(part 1 of 2)
# Autodesk Inventor assembly: DesignRootModel^PCB_ESP32-C3-MINI-1_V1(2)_PCB_ESP32-C3-MINI-1_V1
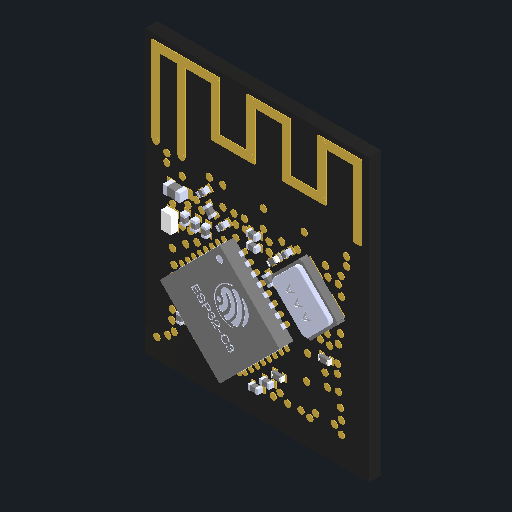
[picture p0: Inventor's stored thumbnail of the model, 512x512]
Saved by Autodesk Inventor 2026.2 (Build 302298000, 298)
## iProperties
Created: 2025-12-23
Part Number: DesignRootModel^PCB_ESP32-C3-MINI-1_V1(2)_PCB_ESP32-C3-MINI-1_V1
Document SubType Name: Assembly
Designer: test
Author: test
## Documents named in this file (333)
- D:\Projects\WearableWLED\WearableWLED_Mechanical\board\WearableWLED_Hardware\WearableWLED_Hardware\DesignRootModel^PCB_ESP32-C3-MINI-1_V1(2)_PCB_ESP32-C3-MINI-1_V1.iam
- D:\Projects\WearableWLED\WearableWLED_Mechanical\board\WearableWLED_Hardware\WearableWLED_Hardware\Submodel-SOD882_part^DesignRootModel_PCB_ESP32-C3-MINI-1_V1(2)_PCB_ESP32-C3-MINI-1_V1.iam
- D:\Projects\WearableWLED\WearableWLED_Mechanical\board\WearableWLED_Hardware\WearableWLED_Hardware\Submodel-R0201_part^DesignRootModel_PCB_ESP32-C3-MINI-1_V1(2)_PCB_ESP32-C3-MINI-1_V1.iam
- D:\Projects\WearableWLED\WearableWLED_Mechanical\board\WearableWLED_Hardware\WearableWLED_Hardware\Submodel-MINI-ANT-TYPED-H_1968823293_part^DesignRootModel_PCB_ESP32-C3-MINI-1_V1(2)_PCB_ESP32-C3-MIN.iam
- D:\Projects\WearableWLED\WearableWLED_Mechanical\board\WearableWLED_Hardware\WearableWLED_Hardware\Submodel-C0402_part^DesignRootModel_PCB_ESP32-C3-MINI-1_V1(2)_PCB_ESP32-C3-MINI-1_V1.iam
- D:\Projects\WearableWLED\WearableWLED_Mechanical\board\WearableWLED_Hardware\WearableWLED_Hardware\Submodel-R0201_part^DesignRootModel_PCB_ESP32-C3-MINI-1_V1(2)_PCB_ESP32-C3-MINI-1_V1_1.iam
- D:\Projects\WearableWLED\WearableWLED_Mechanical\board\WearableWLED_Hardware\WearableWLED_Hardware\Submodel-C0201_part^DesignRootModel_PCB_ESP32-C3-MINI-1_V1(2)_PCB_ESP32-C3-MINI-1_V1.iam
- D:\Projects\WearableWLED\WearableWLED_Mechanical\board\WearableWLED_Hardware\WearableWLED_Hardware\Submodel-R0201_part^DesignRootModel_PCB_ESP32-C3-MINI-1_V1(2)_PCB_ESP32-C3-MINI-1_V1_2.iam
- D:\Projects\WearableWLED\WearableWLED_Mechanical\board\WearableWLED_Hardware\WearableWLED_Hardware\Submodel-C0201_part^DesignRootModel_PCB_ESP32-C3-MINI-1_V1(2)_PCB_ESP32-C3-MINI-1_V1_1.iam
- D:\Projects\WearableWLED\WearableWLED_Mechanical\board\WearableWLED_Hardware\WearableWLED_Hardware\Submodel-C0201_part^DesignRootModel_PCB_ESP32-C3-MINI-1_V1(2)_PCB_ESP32-C3-MINI-1_V1_2.iam
- D:\Projects\WearableWLED\WearableWLED_Mechanical\board\WearableWLED_Hardware\WearableWLED_Hardware\Submodel-C0201_part^DesignRootModel_PCB_ESP32-C3-MINI-1_V1(2)_PCB_ESP32-C3-MINI-1_V1_3.iam
- D:\Projects\WearableWLED\WearableWLED_Mechanical\board\WearableWLED_Hardware\WearableWLED_Hardware\Submodel-C0201_part^DesignRootModel_PCB_ESP32-C3-MINI-1_V1(2)_PCB_ESP32-C3-MINI-1_V1_4.iam
- D:\Projects\WearableWLED\WearableWLED_Mechanical\board\WearableWLED_Hardware\WearableWLED_Hardware\Submodel-C0201_part^DesignRootModel_PCB_ESP32-C3-MINI-1_V1(2)_PCB_ESP32-C3-MINI-1_V1_5.iam
- D:\Projects\WearableWLED\WearableWLED_Mechanical\board\WearableWLED_Hardware\WearableWLED_Hardware\Submodel-C0201_part^DesignRootModel_PCB_ESP32-C3-MINI-1_V1(2)_PCB_ESP32-C3-MINI-1_V1_6.iam
- D:\Projects\WearableWLED\WearableWLED_Mechanical\board\WearableWLED_Hardware\WearableWLED_Hardware\Submodel-C0201_part^DesignRootModel_PCB_ESP32-C3-MINI-1_V1(2)_PCB_ESP32-C3-MINI-1_V1_7.iam
- D:\Projects\WearableWLED\WearableWLED_Mechanical\board\WearableWLED_Hardware\WearableWLED_Hardware\Submodel-C0201_part^DesignRootModel_PCB_ESP32-C3-MINI-1_V1(2)_PCB_ESP32-C3-MINI-1_V1_8.iam
- D:\Projects\WearableWLED\WearableWLED_Mechanical\board\WearableWLED_Hardware\WearableWLED_Hardware\Submodel-C0201_part^DesignRootModel_PCB_ESP32-C3-MINI-1_V1(2)_PCB_ESP32-C3-MINI-1_V1_9.iam
- D:\Projects\WearableWLED\WearableWLED_Mechanical\board\WearableWLED_Hardware\WearableWLED_Hardware\Submodel-L0201_part^DesignRootModel_PCB_ESP32-C3-MINI-1_V1(2)_PCB_ESP32-C3-MINI-1_V1.iam
- D:\Projects\WearableWLED\WearableWLED_Mechanical\board\WearableWLED_Hardware\WearableWLED_Hardware\Submodel-L0201_part^DesignRootModel_PCB_ESP32-C3-MINI-1_V1(2)_PCB_ESP32-C3-MINI-1_V1_1.iam
- D:\Projects\WearableWLED\WearableWLED_Mechanical\board\WearableWLED_Hardware\WearableWLED_Hardware\Submodel-XTAL3225_part^DesignRootModel_PCB_ESP32-C3-MINI-1_V1(2)_PCB_ESP32-C3-MINI-1_V1.iam
- D:\Projects\WearableWLED\WearableWLED_Mechanical\board\WearableWLED_Hardware\WearableWLED_Hardware\Submodel-QFN32_0P5_5_part^DesignRootModel_PCB_ESP32-C3-MINI-1_V1(2)_PCB_ESP32-C3-MINI-1_V1.iam
- D:\Projects\WearableWLED\WearableWLED_Mechanical\board\WearableWLED_Hardware\WearableWLED_Hardware\Submodel-C0201_part^DesignRootModel_PCB_ESP32-C3-MINI-1_V1(2)_PCB_ESP32-C3-MINI-1_V1_10.iam
- D:\Projects\WearableWLED\WearableWLED_Mechanical\board\WearableWLED_Hardware\WearableWLED_Hardware\uid__4^DesignRootModel_PCB_ESP32-C3-MINI-1_V1(2)_PCB_ESP32-C3-MINI-1_V1.ipt
- D:\Projects\WearableWLED\WearableWLED_Mechanical\board\WearableWLED_Hardware\WearableWLED_Hardware\uid__4-22^DesignRootModel_PCB_ESP32-C3-MINI-1_V1(2)_PCB_ESP32-C3-MINI-1_V1.ipt
- D:\Projects\WearableWLED\WearableWLED_Mechanical\board\WearableWLED_Hardware\WearableWLED_Hardware\uid__4-23^DesignRootModel_PCB_ESP32-C3-MINI-1_V1(2)_PCB_ESP32-C3-MINI-1_V1.ipt
- D:\Projects\WearableWLED\WearableWLED_Mechanical\board\WearableWLED_Hardware\WearableWLED_Hardware\uid__4-24^DesignRootModel_PCB_ESP32-C3-MINI-1_V1(2)_PCB_ESP32-C3-MINI-1_V1.ipt
- D:\Projects\WearableWLED\WearableWLED_Mechanical\board\WearableWLED_Hardware\WearableWLED_Hardware\uid__4-25^DesignRootModel_PCB_ESP32-C3-MINI-1_V1(2)_PCB_ESP32-C3-MINI-1_V1.ipt
- D:\Projects\WearableWLED\WearableWLED_Mechanical\board\WearableWLED_Hardware\WearableWLED_Hardware\uid__4-26^DesignRootModel_PCB_ESP32-C3-MINI-1_V1(2)_PCB_ESP32-C3-MINI-1_V1.ipt
- D:\Projects\WearableWLED\WearableWLED_Mechanical\board\WearableWLED_Hardware\WearableWLED_Hardware\uid__4-27^DesignRootModel_PCB_ESP32-C3-MINI-1_V1(2)_PCB_ESP32-C3-MINI-1_V1.ipt
- D:\Projects\WearableWLED\WearableWLED_Mechanical\board\WearableWLED_Hardware\WearableWLED_Hardware\uid__4-28^DesignRootModel_PCB_ESP32-C3-MINI-1_V1(2)_PCB_ESP32-C3-MINI-1_V1.ipt
- D:\Projects\WearableWLED\WearableWLED_Mechanical\board\WearableWLED_Hardware\WearableWLED_Hardware\uid__4-29^DesignRootModel_PCB_ESP32-C3-MINI-1_V1(2)_PCB_ESP32-C3-MINI-1_V1.ipt
- D:\Projects\WearableWLED\WearableWLED_Mechanical\board\WearableWLED_Hardware\WearableWLED_Hardware\uid__4-30^DesignRootModel_PCB_ESP32-C3-MINI-1_V1(2)_PCB_ESP32-C3-MINI-1_V1.ipt
- D:\Projects\WearableWLED\WearableWLED_Mechanical\board\WearableWLED_Hardware\WearableWLED_Hardware\uid__4-31^DesignRootModel_PCB_ESP32-C3-MINI-1_V1(2)_PCB_ESP32-C3-MINI-1_V1.ipt
- D:\Projects\WearableWLED\WearableWLED_Mechanical\board\WearableWLED_Hardware\WearableWLED_Hardware\uid__4-32^DesignRootModel_PCB_ESP32-C3-MINI-1_V1(2)_PCB_ESP32-C3-MINI-1_V1.ipt
- D:\Projects\WearableWLED\WearableWLED_Mechanical\board\WearableWLED_Hardware\WearableWLED_Hardware\uid__4-33^DesignRootModel_PCB_ESP32-C3-MINI-1_V1(2)_PCB_ESP32-C3-MINI-1_V1.ipt
- D:\Projects\WearableWLED\WearableWLED_Mechanical\board\WearableWLED_Hardware\WearableWLED_Hardware\uid__4-34^DesignRootModel_PCB_ESP32-C3-MINI-1_V1(2)_PCB_ESP32-C3-MINI-1_V1.ipt
- D:\Projects\WearableWLED\WearableWLED_Mechanical\board\WearableWLED_Hardware\WearableWLED_Hardware\uid__4-35^DesignRootModel_PCB_ESP32-C3-MINI-1_V1(2)_PCB_ESP32-C3-MINI-1_V1.ipt
- D:\Projects\WearableWLED\WearableWLED_Mechanical\board\WearableWLED_Hardware\WearableWLED_Hardware\uid__4-36^DesignRootModel_PCB_ESP32-C3-MINI-1_V1(2)_PCB_ESP32-C3-MINI-1_V1.ipt
- D:\Projects\WearableWLED\WearableWLED_Mechanical\board\WearableWLED_Hardware\WearableWLED_Hardware\uid__4-37^DesignRootModel_PCB_ESP32-C3-MINI-1_V1(2)_PCB_ESP32-C3-MINI-1_V1.ipt
- D:\Projects\WearableWLED\WearableWLED_Mechanical\board\WearableWLED_Hardware\WearableWLED_Hardware\uid__4-38^DesignRootModel_PCB_ESP32-C3-MINI-1_V1(2)_PCB_ESP32-C3-MINI-1_V1.ipt
- D:\Projects\WearableWLED\WearableWLED_Mechanical\board\WearableWLED_Hardware\WearableWLED_Hardware\uid__4-39^DesignRootModel_PCB_ESP32-C3-MINI-1_V1(2)_PCB_ESP32-C3-MINI-1_V1.ipt
- D:\Projects\WearableWLED\WearableWLED_Mechanical\board\WearableWLED_Hardware\WearableWLED_Hardware\uid__4-40^DesignRootModel_PCB_ESP32-C3-MINI-1_V1(2)_PCB_ESP32-C3-MINI-1_V1.ipt
- D:\Projects\WearableWLED\WearableWLED_Mechanical\board\WearableWLED_Hardware\WearableWLED_Hardware\uid__4-41^DesignRootModel_PCB_ESP32-C3-MINI-1_V1(2)_PCB_ESP32-C3-MINI-1_V1.ipt
- D:\Projects\WearableWLED\WearableWLED_Mechanical\board\WearableWLED_Hardware\WearableWLED_Hardware\uid__4-42^DesignRootModel_PCB_ESP32-C3-MINI-1_V1(2)_PCB_ESP32-C3-MINI-1_V1.ipt
- D:\Projects\WearableWLED\WearableWLED_Mechanical\board\WearableWLED_Hardware\WearableWLED_Hardware\uid__4-43^DesignRootModel_PCB_ESP32-C3-MINI-1_V1(2)_PCB_ESP32-C3-MINI-1_V1.ipt
- D:\Projects\WearableWLED\WearableWLED_Mechanical\board\WearableWLED_Hardware\WearableWLED_Hardware\uid__4-44^DesignRootModel_PCB_ESP32-C3-MINI-1_V1(2)_PCB_ESP32-C3-MINI-1_V1.ipt
- D:\Projects\WearableWLED\WearableWLED_Mechanical\board\WearableWLED_Hardware\WearableWLED_Hardware\uid__4-45^DesignRootModel_PCB_ESP32-C3-MINI-1_V1(2)_PCB_ESP32-C3-MINI-1_V1.ipt
- D:\Projects\WearableWLED\WearableWLED_Mechanical\board\WearableWLED_Hardware\WearableWLED_Hardware\uid__4-46^DesignRootModel_PCB_ESP32-C3-MINI-1_V1(2)_PCB_ESP32-C3-MINI-1_V1.ipt
- D:\Projects\WearableWLED\WearableWLED_Mechanical\board\WearableWLED_Hardware\WearableWLED_Hardware\uid__4-47^DesignRootModel_PCB_ESP32-C3-MINI-1_V1(2)_PCB_ESP32-C3-MINI-1_V1.ipt
- D:\Projects\WearableWLED\WearableWLED_Mechanical\board\WearableWLED_Hardware\WearableWLED_Hardware\uid__4-48^DesignRootModel_PCB_ESP32-C3-MINI-1_V1(2)_PCB_ESP32-C3-MINI-1_V1.ipt
- D:\Projects\WearableWLED\WearableWLED_Mechanical\board\WearableWLED_Hardware\WearableWLED_Hardware\uid__4-49^DesignRootModel_PCB_ESP32-C3-MINI-1_V1(2)_PCB_ESP32-C3-MINI-1_V1.ipt
- D:\Projects\WearableWLED\WearableWLED_Mechanical\board\WearableWLED_Hardware\WearableWLED_Hardware\uid__4-50^DesignRootModel_PCB_ESP32-C3-MINI-1_V1(2)_PCB_ESP32-C3-MINI-1_V1.ipt
- D:\Projects\WearableWLED\WearableWLED_Mechanical\board\WearableWLED_Hardware\WearableWLED_Hardware\uid__4-51^DesignRootModel_PCB_ESP32-C3-MINI-1_V1(2)_PCB_ESP32-C3-MINI-1_V1.ipt
- D:\Projects\WearableWLED\WearableWLED_Mechanical\board\WearableWLED_Hardware\WearableWLED_Hardware\uid__4-52^DesignRootModel_PCB_ESP32-C3-MINI-1_V1(2)_PCB_ESP32-C3-MINI-1_V1.ipt
- D:\Projects\WearableWLED\WearableWLED_Mechanical\board\WearableWLED_Hardware\WearableWLED_Hardware\uid__4-53^DesignRootModel_PCB_ESP32-C3-MINI-1_V1(2)_PCB_ESP32-C3-MINI-1_V1.ipt
- D:\Projects\WearableWLED\WearableWLED_Mechanical\board\WearableWLED_Hardware\WearableWLED_Hardware\uid__4-54^DesignRootModel_PCB_ESP32-C3-MINI-1_V1(2)_PCB_ESP32-C3-MINI-1_V1.ipt
- D:\Projects\WearableWLED\WearableWLED_Mechanical\board\WearableWLED_Hardware\WearableWLED_Hardware\uid__4-55^DesignRootModel_PCB_ESP32-C3-MINI-1_V1(2)_PCB_ESP32-C3-MINI-1_V1.ipt
- D:\Projects\WearableWLED\WearableWLED_Mechanical\board\WearableWLED_Hardware\WearableWLED_Hardware\uid__4-56^DesignRootModel_PCB_ESP32-C3-MINI-1_V1(2)_PCB_ESP32-C3-MINI-1_V1.ipt
- D:\Projects\WearableWLED\WearableWLED_Mechanical\board\WearableWLED_Hardware\WearableWLED_Hardware\uid__4-57^DesignRootModel_PCB_ESP32-C3-MINI-1_V1(2)_PCB_ESP32-C3-MINI-1_V1.ipt
- D:\Projects\WearableWLED\WearableWLED_Mechanical\board\WearableWLED_Hardware\WearableWLED_Hardware\uid__4-58^DesignRootModel_PCB_ESP32-C3-MINI-1_V1(2)_PCB_ESP32-C3-MINI-1_V1.ipt
- D:\Projects\WearableWLED\WearableWLED_Mechanical\board\WearableWLED_Hardware\WearableWLED_Hardware\uid__4-59^DesignRootModel_PCB_ESP32-C3-MINI-1_V1(2)_PCB_ESP32-C3-MINI-1_V1.ipt
- D:\Projects\WearableWLED\WearableWLED_Mechanical\board\WearableWLED_Hardware\WearableWLED_Hardware\uid__4-60^DesignRootModel_PCB_ESP32-C3-MINI-1_V1(2)_PCB_ESP32-C3-MINI-1_V1.ipt
- D:\Projects\WearableWLED\WearableWLED_Mechanical\board\WearableWLED_Hardware\WearableWLED_Hardware\uid__4-61^DesignRootModel_PCB_ESP32-C3-MINI-1_V1(2)_PCB_ESP32-C3-MINI-1_V1.ipt
- D:\Projects\WearableWLED\WearableWLED_Mechanical\board\WearableWLED_Hardware\WearableWLED_Hardware\uid__4-62^DesignRootModel_PCB_ESP32-C3-MINI-1_V1(2)_PCB_ESP32-C3-MINI-1_V1.ipt
- D:\Projects\WearableWLED\WearableWLED_Mechanical\board\WearableWLED_Hardware\WearableWLED_Hardware\uid__4-63^DesignRootModel_PCB_ESP32-C3-MINI-1_V1(2)_PCB_ESP32-C3-MINI-1_V1.ipt
- D:\Projects\WearableWLED\WearableWLED_Mechanical\board\WearableWLED_Hardware\WearableWLED_Hardware\uid__4-64^DesignRootModel_PCB_ESP32-C3-MINI-1_V1(2)_PCB_ESP32-C3-MINI-1_V1.ipt
- D:\Projects\WearableWLED\WearableWLED_Mechanical\board\WearableWLED_Hardware\WearableWLED_Hardware\uid__4-65^DesignRootModel_PCB_ESP32-C3-MINI-1_V1(2)_PCB_ESP32-C3-MINI-1_V1.ipt
- D:\Projects\WearableWLED\WearableWLED_Mechanical\board\WearableWLED_Hardware\WearableWLED_Hardware\uid__4-66^DesignRootModel_PCB_ESP32-C3-MINI-1_V1(2)_PCB_ESP32-C3-MINI-1_V1.ipt
- D:\Projects\WearableWLED\WearableWLED_Mechanical\board\WearableWLED_Hardware\WearableWLED_Hardware\uid__4-67^DesignRootModel_PCB_ESP32-C3-MINI-1_V1(2)_PCB_ESP32-C3-MINI-1_V1.ipt
- D:\Projects\WearableWLED\WearableWLED_Mechanical\board\WearableWLED_Hardware\WearableWLED_Hardware\uid__4-68^DesignRootModel_PCB_ESP32-C3-MINI-1_V1(2)_PCB_ESP32-C3-MINI-1_V1.ipt
- D:\Projects\WearableWLED\WearableWLED_Mechanical\board\WearableWLED_Hardware\WearableWLED_Hardware\uid__4-69^DesignRootModel_PCB_ESP32-C3-MINI-1_V1(2)_PCB_ESP32-C3-MINI-1_V1.ipt
- D:\Projects\WearableWLED\WearableWLED_Mechanical\board\WearableWLED_Hardware\WearableWLED_Hardware\uid__4-70^DesignRootModel_PCB_ESP32-C3-MINI-1_V1(2)_PCB_ESP32-C3-MINI-1_V1.ipt
- D:\Projects\WearableWLED\WearableWLED_Mechanical\board\WearableWLED_Hardware\WearableWLED_Hardware\uid__4-71^DesignRootModel_PCB_ESP32-C3-MINI-1_V1(2)_PCB_ESP32-C3-MINI-1_V1.ipt
- D:\Projects\WearableWLED\WearableWLED_Mechanical\board\WearableWLED_Hardware\WearableWLED_Hardware\uid__4-72^DesignRootModel_PCB_ESP32-C3-MINI-1_V1(2)_PCB_ESP32-C3-MINI-1_V1.ipt
- D:\Projects\WearableWLED\WearableWLED_Mechanical\board\WearableWLED_Hardware\WearableWLED_Hardware\uid__4-73^DesignRootModel_PCB_ESP32-C3-MINI-1_V1(2)_PCB_ESP32-C3-MINI-1_V1.ipt
- D:\Projects\WearableWLED\WearableWLED_Mechanical\board\WearableWLED_Hardware\WearableWLED_Hardware\uid__4-74^DesignRootModel_PCB_ESP32-C3-MINI-1_V1(2)_PCB_ESP32-C3-MINI-1_V1.ipt
- D:\Projects\WearableWLED\WearableWLED_Mechanical\board\WearableWLED_Hardware\WearableWLED_Hardware\uid__4-75^DesignRootModel_PCB_ESP32-C3-MINI-1_V1(2)_PCB_ESP32-C3-MINI-1_V1.ipt
- D:\Projects\WearableWLED\WearableWLED_Mechanical\board\WearableWLED_Hardware\WearableWLED_Hardware\uid__4-76^DesignRootModel_PCB_ESP32-C3-MINI-1_V1(2)_PCB_ESP32-C3-MINI-1_V1.ipt
- D:\Projects\WearableWLED\WearableWLED_Mechanical\board\WearableWLED_Hardware\WearableWLED_Hardware\uid__4-77^DesignRootModel_PCB_ESP32-C3-MINI-1_V1(2)_PCB_ESP32-C3-MINI-1_V1.ipt
- D:\Projects\WearableWLED\WearableWLED_Mechanical\board\WearableWLED_Hardware\WearableWLED_Hardware\uid__4-78^DesignRootModel_PCB_ESP32-C3-MINI-1_V1(2)_PCB_ESP32-C3-MINI-1_V1.ipt
- D:\Projects\WearableWLED\WearableWLED_Mechanical\board\WearableWLED_Hardware\WearableWLED_Hardware\uid__4-79^DesignRootModel_PCB_ESP32-C3-MINI-1_V1(2)_PCB_ESP32-C3-MINI-1_V1.ipt
- D:\Projects\WearableWLED\WearableWLED_Mechanical\board\WearableWLED_Hardware\WearableWLED_Hardware\uid__4-80^DesignRootModel_PCB_ESP32-C3-MINI-1_V1(2)_PCB_ESP32-C3-MINI-1_V1.ipt
- D:\Projects\WearableWLED\WearableWLED_Mechanical\board\WearableWLED_Hardware\WearableWLED_Hardware\uid__4-81^DesignRootModel_PCB_ESP32-C3-MINI-1_V1(2)_PCB_ESP32-C3-MINI-1_V1.ipt
- D:\Projects\WearableWLED\WearableWLED_Mechanical\board\WearableWLED_Hardware\WearableWLED_Hardware\uid__4-82^DesignRootModel_PCB_ESP32-C3-MINI-1_V1(2)_PCB_ESP32-C3-MINI-1_V1.ipt
- D:\Projects\WearableWLED\WearableWLED_Mechanical\board\WearableWLED_Hardware\WearableWLED_Hardware\uid__4-83^DesignRootModel_PCB_ESP32-C3-MINI-1_V1(2)_PCB_ESP32-C3-MINI-1_V1.ipt
- D:\Projects\WearableWLED\WearableWLED_Mechanical\board\WearableWLED_Hardware\WearableWLED_Hardware\uid__4-84^DesignRootModel_PCB_ESP32-C3-MINI-1_V1(2)_PCB_ESP32-C3-MINI-1_V1.ipt
- D:\Projects\WearableWLED\WearableWLED_Mechanical\board\WearableWLED_Hardware\WearableWLED_Hardware\uid__4-85^DesignRootModel_PCB_ESP32-C3-MINI-1_V1(2)_PCB_ESP32-C3-MINI-1_V1.ipt
- D:\Projects\WearableWLED\WearableWLED_Mechanical\board\WearableWLED_Hardware\WearableWLED_Hardware\uid__4-86^DesignRootModel_PCB_ESP32-C3-MINI-1_V1(2)_PCB_ESP32-C3-MINI-1_V1.ipt
- D:\Projects\WearableWLED\WearableWLED_Mechanical\board\WearableWLED_Hardware\WearableWLED_Hardware\uid__4-87^DesignRootModel_PCB_ESP32-C3-MINI-1_V1(2)_PCB_ESP32-C3-MINI-1_V1.ipt
- D:\Projects\WearableWLED\WearableWLED_Mechanical\board\WearableWLED_Hardware\WearableWLED_Hardware\uid__4-88^DesignRootModel_PCB_ESP32-C3-MINI-1_V1(2)_PCB_ESP32-C3-MINI-1_V1.ipt
- D:\Projects\WearableWLED\WearableWLED_Mechanical\board\WearableWLED_Hardware\WearableWLED_Hardware\uid__4-89^DesignRootModel_PCB_ESP32-C3-MINI-1_V1(2)_PCB_ESP32-C3-MINI-1_V1.ipt
- D:\Projects\WearableWLED\WearableWLED_Mechanical\board\WearableWLED_Hardware\WearableWLED_Hardware\uid__4-90^DesignRootModel_PCB_ESP32-C3-MINI-1_V1(2)_PCB_ESP32-C3-MINI-1_V1.ipt
- D:\Projects\WearableWLED\WearableWLED_Mechanical\board\WearableWLED_Hardware\WearableWLED_Hardware\uid__4-91^DesignRootModel_PCB_ESP32-C3-MINI-1_V1(2)_PCB_ESP32-C3-MINI-1_V1.ipt
- D:\Projects\WearableWLED\WearableWLED_Mechanical\board\WearableWLED_Hardware\WearableWLED_Hardware\uid__4-92^DesignRootModel_PCB_ESP32-C3-MINI-1_V1(2)_PCB_ESP32-C3-MINI-1_V1.ipt
- D:\Projects\WearableWLED\WearableWLED_Mechanical\board\WearableWLED_Hardware\WearableWLED_Hardware\uid__4-93^DesignRootModel_PCB_ESP32-C3-MINI-1_V1(2)_PCB_ESP32-C3-MINI-1_V1.ipt
- D:\Projects\WearableWLED\WearableWLED_Mechanical\board\WearableWLED_Hardware\WearableWLED_Hardware\uid__4-94^DesignRootModel_PCB_ESP32-C3-MINI-1_V1(2)_PCB_ESP32-C3-MINI-1_V1.ipt
- D:\Projects\WearableWLED\WearableWLED_Mechanical\board\WearableWLED_Hardware\WearableWLED_Hardware\uid__4-95^DesignRootModel_PCB_ESP32-C3-MINI-1_V1(2)_PCB_ESP32-C3-MINI-1_V1.ipt
- D:\Projects\WearableWLED\WearableWLED_Mechanical\board\WearableWLED_Hardware\WearableWLED_Hardware\uid__4-96^DesignRootModel_PCB_ESP32-C3-MINI-1_V1(2)_PCB_ESP32-C3-MINI-1_V1.ipt
- D:\Projects\WearableWLED\WearableWLED_Mechanical\board\WearableWLED_Hardware\WearableWLED_Hardware\uid__4-97^DesignRootModel_PCB_ESP32-C3-MINI-1_V1(2)_PCB_ESP32-C3-MINI-1_V1.ipt
- D:\Projects\WearableWLED\WearableWLED_Mechanical\board\WearableWLED_Hardware\WearableWLED_Hardware\uid__4-98^DesignRootModel_PCB_ESP32-C3-MINI-1_V1(2)_PCB_ESP32-C3-MINI-1_V1.ipt
- D:\Projects\WearableWLED\WearableWLED_Mechanical\board\WearableWLED_Hardware\WearableWLED_Hardware\uid__4-99^DesignRootModel_PCB_ESP32-C3-MINI-1_V1(2)_PCB_ESP32-C3-MINI-1_V1.ipt
- D:\Projects\WearableWLED\WearableWLED_Mechanical\board\WearableWLED_Hardware\WearableWLED_Hardware\uid__4-100^DesignRootModel_PCB_ESP32-C3-MINI-1_V1(2)_PCB_ESP32-C3-MINI-1_V1.ipt
- D:\Projects\WearableWLED\WearableWLED_Mechanical\board\WearableWLED_Hardware\WearableWLED_Hardware\uid__4-101^DesignRootModel_PCB_ESP32-C3-MINI-1_V1(2)_PCB_ESP32-C3-MINI-1_V1.ipt
- D:\Projects\WearableWLED\WearableWLED_Mechanical\board\WearableWLED_Hardware\WearableWLED_Hardware\uid__4-102^DesignRootModel_PCB_ESP32-C3-MINI-1_V1(2)_PCB_ESP32-C3-MINI-1_V1.ipt
- D:\Projects\WearableWLED\WearableWLED_Mechanical\board\WearableWLED_Hardware\WearableWLED_Hardware\uid__4-103^DesignRootModel_PCB_ESP32-C3-MINI-1_V1(2)_PCB_ESP32-C3-MINI-1_V1.ipt
- D:\Projects\WearableWLED\WearableWLED_Mechanical\board\WearableWLED_Hardware\WearableWLED_Hardware\uid__4-104^DesignRootModel_PCB_ESP32-C3-MINI-1_V1(2)_PCB_ESP32-C3-MINI-1_V1.ipt
- D:\Projects\WearableWLED\WearableWLED_Mechanical\board\WearableWLED_Hardware\WearableWLED_Hardware\uid__4-105^DesignRootModel_PCB_ESP32-C3-MINI-1_V1(2)_PCB_ESP32-C3-MINI-1_V1.ipt
- D:\Projects\WearableWLED\WearableWLED_Mechanical\board\WearableWLED_Hardware\WearableWLED_Hardware\uid__4-106^DesignRootModel_PCB_ESP32-C3-MINI-1_V1(2)_PCB_ESP32-C3-MINI-1_V1.ipt
- D:\Projects\WearableWLED\WearableWLED_Mechanical\board\WearableWLED_Hardware\WearableWLED_Hardware\uid__4-107^DesignRootModel_PCB_ESP32-C3-MINI-1_V1(2)_PCB_ESP32-C3-MINI-1_V1.ipt
- D:\Projects\WearableWLED\WearableWLED_Mechanical\board\WearableWLED_Hardware\WearableWLED_Hardware\uid__4-108^DesignRootModel_PCB_ESP32-C3-MINI-1_V1(2)_PCB_ESP32-C3-MINI-1_V1.ipt
- D:\Projects\WearableWLED\WearableWLED_Mechanical\board\WearableWLED_Hardware\WearableWLED_Hardware\uid__4-109^DesignRootModel_PCB_ESP32-C3-MINI-1_V1(2)_PCB_ESP32-C3-MINI-1_V1.ipt
- D:\Projects\WearableWLED\WearableWLED_Mechanical\board\WearableWLED_Hardware\WearableWLED_Hardware\uid__4-110^DesignRootModel_PCB_ESP32-C3-MINI-1_V1(2)_PCB_ESP32-C3-MINI-1_V1.ipt
- D:\Projects\WearableWLED\WearableWLED_Mechanical\board\WearableWLED_Hardware\WearableWLED_Hardware\uid__4-111^DesignRootModel_PCB_ESP32-C3-MINI-1_V1(2)_PCB_ESP32-C3-MINI-1_V1.ipt
- D:\Projects\WearableWLED\WearableWLED_Mechanical\board\WearableWLED_Hardware\WearableWLED_Hardware\uid__4-112^DesignRootModel_PCB_ESP32-C3-MINI-1_V1(2)_PCB_ESP32-C3-MINI-1_V1.ipt
- D:\Projects\WearableWLED\WearableWLED_Mechanical\board\WearableWLED_Hardware\WearableWLED_Hardware\uid__4-113^DesignRootModel_PCB_ESP32-C3-MINI-1_V1(2)_PCB_ESP32-C3-MINI-1_V1.ipt
- D:\Projects\WearableWLED\WearableWLED_Mechanical\board\WearableWLED_Hardware\WearableWLED_Hardware\uid__4-114^DesignRootModel_PCB_ESP32-C3-MINI-1_V1(2)_PCB_ESP32-C3-MINI-1_V1.ipt
- D:\Projects\WearableWLED\WearableWLED_Mechanical\board\WearableWLED_Hardware\WearableWLED_Hardware\uid__4-115^DesignRootModel_PCB_ESP32-C3-MINI-1_V1(2)_PCB_ESP32-C3-MINI-1_V1.ipt
- D:\Projects\WearableWLED\WearableWLED_Mechanical\board\WearableWLED_Hardware\WearableWLED_Hardware\uid__4-116^DesignRootModel_PCB_ESP32-C3-MINI-1_V1(2)_PCB_ESP32-C3-MINI-1_V1.ipt
- D:\Projects\WearableWLED\WearableWLED_Mechanical\board\WearableWLED_Hardware\WearableWLED_Hardware\uid__4-117^DesignRootModel_PCB_ESP32-C3-MINI-1_V1(2)_PCB_ESP32-C3-MINI-1_V1.ipt
- D:\Projects\WearableWLED\WearableWLED_Mechanical\board\WearableWLED_Hardware\WearableWLED_Hardware\uid__4-118^DesignRootModel_PCB_ESP32-C3-MINI-1_V1(2)_PCB_ESP32-C3-MINI-1_V1.ipt
- D:\Projects\WearableWLED\WearableWLED_Mechanical\board\WearableWLED_Hardware\WearableWLED_Hardware\uid__4-119^DesignRootModel_PCB_ESP32-C3-MINI-1_V1(2)_PCB_ESP32-C3-MINI-1_V1.ipt
- D:\Projects\WearableWLED\WearableWLED_Mechanical\board\WearableWLED_Hardware\WearableWLED_Hardware\uid__4-120^DesignRootModel_PCB_ESP32-C3-MINI-1_V1(2)_PCB_ESP32-C3-MINI-1_V1.ipt
- D:\Projects\WearableWLED\WearableWLED_Mechanical\board\WearableWLED_Hardware\WearableWLED_Hardware\uid__4-121^DesignRootModel_PCB_ESP32-C3-MINI-1_V1(2)_PCB_ESP32-C3-MINI-1_V1.ipt
- D:\Projects\WearableWLED\WearableWLED_Mechanical\board\WearableWLED_Hardware\WearableWLED_Hardware\uid__4-122^DesignRootModel_PCB_ESP32-C3-MINI-1_V1(2)_PCB_ESP32-C3-MINI-1_V1.ipt
- D:\Projects\WearableWLED\WearableWLED_Mechanical\board\WearableWLED_Hardware\WearableWLED_Hardware\uid__4-123^DesignRootModel_PCB_ESP32-C3-MINI-1_V1(2)_PCB_ESP32-C3-MINI-1_V1.ipt
- D:\Projects\WearableWLED\WearableWLED_Mechanical\board\WearableWLED_Hardware\WearableWLED_Hardware\uid__4-124^DesignRootModel_PCB_ESP32-C3-MINI-1_V1(2)_PCB_ESP32-C3-MINI-1_V1.ipt
- D:\Projects\WearableWLED\WearableWLED_Mechanical\board\WearableWLED_Hardware\WearableWLED_Hardware\uid__4-125^DesignRootModel_PCB_ESP32-C3-MINI-1_V1(2)_PCB_ESP32-C3-MINI-1_V1.ipt
- D:\Projects\WearableWLED\WearableWLED_Mechanical\board\WearableWLED_Hardware\WearableWLED_Hardware\uid__4-126^DesignRootModel_PCB_ESP32-C3-MINI-1_V1(2)_PCB_ESP32-C3-MINI-1_V1.ipt
- D:\Projects\WearableWLED\WearableWLED_Mechanical\board\WearableWLED_Hardware\WearableWLED_Hardware\uid__4-127^DesignRootModel_PCB_ESP32-C3-MINI-1_V1(2)_PCB_ESP32-C3-MINI-1_V1.ipt
- D:\Projects\WearableWLED\WearableWLED_Mechanical\board\WearableWLED_Hardware\WearableWLED_Hardware\uid__4-128^DesignRootModel_PCB_ESP32-C3-MINI-1_V1(2)_PCB_ESP32-C3-MINI-1_V1.ipt
- D:\Projects\WearableWLED\WearableWLED_Mechanical\board\WearableWLED_Hardware\WearableWLED_Hardware\uid__4-129^DesignRootModel_PCB_ESP32-C3-MINI-1_V1(2)_PCB_ESP32-C3-MINI-1_V1.ipt
- D:\Projects\WearableWLED\WearableWLED_Mechanical\board\WearableWLED_Hardware\WearableWLED_Hardware\uid__4-130^DesignRootModel_PCB_ESP32-C3-MINI-1_V1(2)_PCB_ESP32-C3-MINI-1_V1.ipt
- D:\Projects\WearableWLED\WearableWLED_Mechanical\board\WearableWLED_Hardware\WearableWLED_Hardware\uid__4-131^DesignRootModel_PCB_ESP32-C3-MINI-1_V1(2)_PCB_ESP32-C3-MINI-1_V1.ipt
- D:\Projects\WearableWLED\WearableWLED_Mechanical\board\WearableWLED_Hardware\WearableWLED_Hardware\uid__4-132^DesignRootModel_PCB_ESP32-C3-MINI-1_V1(2)_PCB_ESP32-C3-MINI-1_V1.ipt
- D:\Projects\WearableWLED\WearableWLED_Mechanical\board\WearableWLED_Hardware\WearableWLED_Hardware\uid__4-133^DesignRootModel_PCB_ESP32-C3-MINI-1_V1(2)_PCB_ESP32-C3-MINI-1_V1.ipt
- D:\Projects\WearableWLED\WearableWLED_Mechanical\board\WearableWLED_Hardware\WearableWLED_Hardware\uid__4-134^DesignRootModel_PCB_ESP32-C3-MINI-1_V1(2)_PCB_ESP32-C3-MINI-1_V1.ipt
- D:\Projects\WearableWLED\WearableWLED_Mechanical\board\WearableWLED_Hardware\WearableWLED_Hardware\uid__4-135^DesignRootModel_PCB_ESP32-C3-MINI-1_V1(2)_PCB_ESP32-C3-MINI-1_V1.ipt
- D:\Projects\WearableWLED\WearableWLED_Mechanical\board\WearableWLED_Hardware\WearableWLED_Hardware\uid__4-136^DesignRootModel_PCB_ESP32-C3-MINI-1_V1(2)_PCB_ESP32-C3-MINI-1_V1.ipt
- D:\Projects\WearableWLED\WearableWLED_Mechanical\board\WearableWLED_Hardware\WearableWLED_Hardware\uid__4-137^DesignRootModel_PCB_ESP32-C3-MINI-1_V1(2)_PCB_ESP32-C3-MINI-1_V1.ipt
- D:\Projects\WearableWLED\WearableWLED_Mechanical\board\WearableWLED_Hardware\WearableWLED_Hardware\uid__4-138^DesignRootModel_PCB_ESP32-C3-MINI-1_V1(2)_PCB_ESP32-C3-MINI-1_V1.ipt
- D:\Projects\WearableWLED\WearableWLED_Mechanical\board\WearableWLED_Hardware\WearableWLED_Hardware\uid__4-139^DesignRootModel_PCB_ESP32-C3-MINI-1_V1(2)_PCB_ESP32-C3-MINI-1_V1.ipt
- D:\Projects\WearableWLED\WearableWLED_Mechanical\board\WearableWLED_Hardware\WearableWLED_Hardware\uid__4-140^DesignRootModel_PCB_ESP32-C3-MINI-1_V1(2)_PCB_ESP32-C3-MINI-1_V1.ipt
- D:\Projects\WearableWLED\WearableWLED_Mechanical\board\WearableWLED_Hardware\WearableWLED_Hardware\uid__4-141^DesignRootModel_PCB_ESP32-C3-MINI-1_V1(2)_PCB_ESP32-C3-MINI-1_V1.ipt
- D:\Projects\WearableWLED\WearableWLED_Mechanical\board\WearableWLED_Hardware\WearableWLED_Hardware\uid__4-142^DesignRootModel_PCB_ESP32-C3-MINI-1_V1(2)_PCB_ESP32-C3-MINI-1_V1.ipt
- D:\Projects\WearableWLED\WearableWLED_Mechanical\board\WearableWLED_Hardware\WearableWLED_Hardware\uid__4-143^DesignRootModel_PCB_ESP32-C3-MINI-1_V1(2)_PCB_ESP32-C3-MINI-1_V1.ipt
- D:\Projects\WearableWLED\WearableWLED_Mechanical\board\WearableWLED_Hardware\WearableWLED_Hardware\uid__4-144^DesignRootModel_PCB_ESP32-C3-MINI-1_V1(2)_PCB_ESP32-C3-MINI-1_V1.ipt
- D:\Projects\WearableWLED\WearableWLED_Mechanical\board\WearableWLED_Hardware\WearableWLED_Hardware\uid__4-145^DesignRootModel_PCB_ESP32-C3-MINI-1_V1(2)_PCB_ESP32-C3-MINI-1_V1.ipt
- D:\Projects\WearableWLED\WearableWLED_Mechanical\board\WearableWLED_Hardware\WearableWLED_Hardware\uid__4-146^DesignRootModel_PCB_ESP32-C3-MINI-1_V1(2)_PCB_ESP32-C3-MINI-1_V1.ipt
- D:\Projects\WearableWLED\WearableWLED_Mechanical\board\WearableWLED_Hardware\WearableWLED_Hardware\uid__4-147^DesignRootModel_PCB_ESP32-C3-MINI-1_V1(2)_PCB_ESP32-C3-MINI-1_V1.ipt
- D:\Projects\WearableWLED\WearableWLED_Mechanical\board\WearableWLED_Hardware\WearableWLED_Hardware\uid__4-148^DesignRootModel_PCB_ESP32-C3-MINI-1_V1(2)_PCB_ESP32-C3-MINI-1_V1.ipt
- D:\Projects\WearableWLED\WearableWLED_Mechanical\board\WearableWLED_Hardware\WearableWLED_Hardware\uid__4-149^DesignRootModel_PCB_ESP32-C3-MINI-1_V1(2)_PCB_ESP32-C3-MINI-1_V1.ipt
- D:\Projects\WearableWLED\WearableWLED_Mechanical\board\WearableWLED_Hardware\WearableWLED_Hardware\uid__4-150^DesignRootModel_PCB_ESP32-C3-MINI-1_V1(2)_PCB_ESP32-C3-MINI-1_V1.ipt
- D:\Projects\WearableWLED\WearableWLED_Mechanical\board\WearableWLED_Hardware\WearableWLED_Hardware\uid__4-151^DesignRootModel_PCB_ESP32-C3-MINI-1_V1(2)_PCB_ESP32-C3-MINI-1_V1.ipt
- D:\Projects\WearableWLED\WearableWLED_Mechanical\board\WearableWLED_Hardware\WearableWLED_Hardware\uid__4-152^DesignRootModel_PCB_ESP32-C3-MINI-1_V1(2)_PCB_ESP32-C3-MINI-1_V1.ipt
- D:\Projects\WearableWLED\WearableWLED_Mechanical\board\WearableWLED_Hardware\WearableWLED_Hardware\uid__4-153^DesignRootModel_PCB_ESP32-C3-MINI-1_V1(2)_PCB_ESP32-C3-MINI-1_V1.ipt
- D:\Projects\WearableWLED\WearableWLED_Mechanical\board\WearableWLED_Hardware\WearableWLED_Hardware\uid__4-154^DesignRootModel_PCB_ESP32-C3-MINI-1_V1(2)_PCB_ESP32-C3-MINI-1_V1.ipt
- D:\Projects\WearableWLED\WearableWLED_Mechanical\board\WearableWLED_Hardware\WearableWLED_Hardware\uid__4-155^DesignRootModel_PCB_ESP32-C3-MINI-1_V1(2)_PCB_ESP32-C3-MINI-1_V1.ipt
- D:\Projects\WearableWLED\WearableWLED_Mechanical\board\WearableWLED_Hardware\WearableWLED_Hardware\uid__4-156^DesignRootModel_PCB_ESP32-C3-MINI-1_V1(2)_PCB_ESP32-C3-MINI-1_V1.ipt
- D:\Projects\WearableWLED\WearableWLED_Mechanical\board\WearableWLED_Hardware\WearableWLED_Hardware\uid__4-157^DesignRootModel_PCB_ESP32-C3-MINI-1_V1(2)_PCB_ESP32-C3-MINI-1_V1.ipt
- D:\Projects\WearableWLED\WearableWLED_Mechanical\board\WearableWLED_Hardware\WearableWLED_Hardware\uid__4-158^DesignRootModel_PCB_ESP32-C3-MINI-1_V1(2)_PCB_ESP32-C3-MINI-1_V1.ipt
- D:\Projects\WearableWLED\WearableWLED_Mechanical\board\WearableWLED_Hardware\WearableWLED_Hardware\uid__4-159^DesignRootModel_PCB_ESP32-C3-MINI-1_V1(2)_PCB_ESP32-C3-MINI-1_V1.ipt
- D:\Projects\WearableWLED\WearableWLED_Mechanical\board\WearableWLED_Hardware\WearableWLED_Hardware\uid__4-160^DesignRootModel_PCB_ESP32-C3-MINI-1_V1(2)_PCB_ESP32-C3-MINI-1_V1.ipt
- D:\Projects\WearableWLED\WearableWLED_Mechanical\board\WearableWLED_Hardware\WearableWLED_Hardware\uid__1^DesignRootModel_PCB_ESP32-C3-MINI-1_V1(2)_PCB_ESP32-C3-MINI-1_V1.ipt
- D:\Projects\WearableWLED\WearableWLED_Mechanical\board\WearableWLED_Hardware\WearableWLED_Hardware\uid__1-161^DesignRootModel_PCB_ESP32-C3-MINI-1_V1(2)_PCB_ESP32-C3-MINI-1_V1.ipt
- D:\Projects\WearableWLED\WearableWLED_Mechanical\board\WearableWLED_Hardware\WearableWLED_Hardware\uid__1-162^DesignRootModel_PCB_ESP32-C3-MINI-1_V1(2)_PCB_ESP32-C3-MINI-1_V1.ipt
- D:\Projects\WearableWLED\WearableWLED_Mechanical\board\WearableWLED_Hardware\WearableWLED_Hardware\uid__1-163^DesignRootModel_PCB_ESP32-C3-MINI-1_V1(2)_PCB_ESP32-C3-MINI-1_V1.ipt
- D:\Projects\WearableWLED\WearableWLED_Mechanical\board\WearableWLED_Hardware\WearableWLED_Hardware\uid__1-164^DesignRootModel_PCB_ESP32-C3-MINI-1_V1(2)_PCB_ESP32-C3-MINI-1_V1.ipt
- D:\Projects\WearableWLED\WearableWLED_Mechanical\board\WearableWLED_Hardware\WearableWLED_Hardware\uid__1-165^DesignRootModel_PCB_ESP32-C3-MINI-1_V1(2)_PCB_ESP32-C3-MINI-1_V1.ipt
- D:\Projects\WearableWLED\WearableWLED_Mechanical\board\WearableWLED_Hardware\WearableWLED_Hardware\uid__1-166^DesignRootModel_PCB_ESP32-C3-MINI-1_V1(2)_PCB_ESP32-C3-MINI-1_V1.ipt
- D:\Projects\WearableWLED\WearableWLED_Mechanical\board\WearableWLED_Hardware\WearableWLED_Hardware\uid__1-167^DesignRootModel_PCB_ESP32-C3-MINI-1_V1(2)_PCB_ESP32-C3-MINI-1_V1.ipt
- D:\Projects\WearableWLED\WearableWLED_Mechanical\board\WearableWLED_Hardware\WearableWLED_Hardware\uid__1-168^DesignRootModel_PCB_ESP32-C3-MINI-1_V1(2)_PCB_ESP32-C3-MINI-1_V1.ipt
- D:\Projects\WearableWLED\WearableWLED_Mechanical\board\WearableWLED_Hardware\WearableWLED_Hardware\uid__1-169^DesignRootModel_PCB_ESP32-C3-MINI-1_V1(2)_PCB_ESP32-C3-MINI-1_V1.ipt
- D:\Projects\WearableWLED\WearableWLED_Mechanical\board\WearableWLED_Hardware\WearableWLED_Hardware\uid__1-170^DesignRootModel_PCB_ESP32-C3-MINI-1_V1(2)_PCB_ESP32-C3-MINI-1_V1.ipt
- D:\Projects\WearableWLED\WearableWLED_Mechanical\board\WearableWLED_Hardware\WearableWLED_Hardware\uid__1-171^DesignRootModel_PCB_ESP32-C3-MINI-1_V1(2)_PCB_ESP32-C3-MINI-1_V1.ipt
- D:\Projects\WearableWLED\WearableWLED_Mechanical\board\WearableWLED_Hardware\WearableWLED_Hardware\uid__1-172^DesignRootModel_PCB_ESP32-C3-MINI-1_V1(2)_PCB_ESP32-C3-MINI-1_V1.ipt
- D:\Projects\WearableWLED\WearableWLED_Mechanical\board\WearableWLED_Hardware\WearableWLED_Hardware\uid__1-173^DesignRootModel_PCB_ESP32-C3-MINI-1_V1(2)_PCB_ESP32-C3-MINI-1_V1.ipt
- D:\Projects\WearableWLED\WearableWLED_Mechanical\board\WearableWLED_Hardware\WearableWLED_Hardware\uid__1-174^DesignRootModel_PCB_ESP32-C3-MINI-1_V1(2)_PCB_ESP32-C3-MINI-1_V1.ipt
- D:\Projects\WearableWLED\WearableWLED_Mechanical\board\WearableWLED_Hardware\WearableWLED_Hardware\uid__1-175^DesignRootModel_PCB_ESP32-C3-MINI-1_V1(2)_PCB_ESP32-C3-MINI-1_V1.ipt
- D:\Projects\WearableWLED\WearableWLED_Mechanical\board\WearableWLED_Hardware\WearableWLED_Hardware\uid__1-176^DesignRootModel_PCB_ESP32-C3-MINI-1_V1(2)_PCB_ESP32-C3-MINI-1_V1.ipt
- D:\Projects\WearableWLED\WearableWLED_Mechanical\board\WearableWLED_Hardware\WearableWLED_Hardware\uid__1-177^DesignRootModel_PCB_ESP32-C3-MINI-1_V1(2)_PCB_ESP32-C3-MINI-1_V1.ipt
- D:\Projects\WearableWLED\WearableWLED_Mechanical\board\WearableWLED_Hardware\WearableWLED_Hardware\uid__1-178^DesignRootModel_PCB_ESP32-C3-MINI-1_V1(2)_PCB_ESP32-C3-MINI-1_V1.ipt
- D:\Projects\WearableWLED\WearableWLED_Mechanical\board\WearableWLED_Hardware\WearableWLED_Hardware\uid__1-179^DesignRootModel_PCB_ESP32-C3-MINI-1_V1(2)_PCB_ESP32-C3-MINI-1_V1.ipt
- D:\Projects\WearableWLED\WearableWLED_Mechanical\board\WearableWLED_Hardware\WearableWLED_Hardware\uid__1-180^DesignRootModel_PCB_ESP32-C3-MINI-1_V1(2)_PCB_ESP32-C3-MINI-1_V1.ipt
- D:\Projects\WearableWLED\WearableWLED_Mechanical\board\WearableWLED_Hardware\WearableWLED_Hardware\uid__1-181^DesignRootModel_PCB_ESP32-C3-MINI-1_V1(2)_PCB_ESP32-C3-MINI-1_V1.ipt
- D:\Projects\WearableWLED\WearableWLED_Mechanical\board\WearableWLED_Hardware\WearableWLED_Hardware\uid__1-182^DesignRootModel_PCB_ESP32-C3-MINI-1_V1(2)_PCB_ESP32-C3-MINI-1_V1.ipt
- D:\Projects\WearableWLED\WearableWLED_Mechanical\board\WearableWLED_Hardware\WearableWLED_Hardware\uid__1-183^DesignRootModel_PCB_ESP32-C3-MINI-1_V1(2)_PCB_ESP32-C3-MINI-1_V1.ipt
- D:\Projects\WearableWLED\WearableWLED_Mechanical\board\WearableWLED_Hardware\WearableWLED_Hardware\uid__1-184^DesignRootModel_PCB_ESP32-C3-MINI-1_V1(2)_PCB_ESP32-C3-MINI-1_V1.ipt
- D:\Projects\WearableWLED\WearableWLED_Mechanical\board\WearableWLED_Hardware\WearableWLED_Hardware\uid__1-185^DesignRootModel_PCB_ESP32-C3-MINI-1_V1(2)_PCB_ESP32-C3-MINI-1_V1.ipt
- D:\Projects\WearableWLED\WearableWLED_Mechanical\board\WearableWLED_Hardware\WearableWLED_Hardware\uid__1-186^DesignRootModel_PCB_ESP32-C3-MINI-1_V1(2)_PCB_ESP32-C3-MINI-1_V1.ipt
- D:\Projects\WearableWLED\WearableWLED_Mechanical\board\WearableWLED_Hardware\WearableWLED_Hardware\uid__1-187^DesignRootModel_PCB_ESP32-C3-MINI-1_V1(2)_PCB_ESP32-C3-MINI-1_V1.ipt
- D:\Projects\WearableWLED\WearableWLED_Mechanical\board\WearableWLED_Hardware\WearableWLED_Hardware\uid__1-188^DesignRootModel_PCB_ESP32-C3-MINI-1_V1(2)_PCB_ESP32-C3-MINI-1_V1.ipt
- D:\Projects\WearableWLED\WearableWLED_Mechanical\board\WearableWLED_Hardware\WearableWLED_Hardware\uid__1-189^DesignRootModel_PCB_ESP32-C3-MINI-1_V1(2)_PCB_ESP32-C3-MINI-1_V1.ipt
- D:\Projects\WearableWLED\WearableWLED_Mechanical\board\WearableWLED_Hardware\WearableWLED_Hardware\uid__1-190^DesignRootModel_PCB_ESP32-C3-MINI-1_V1(2)_PCB_ESP32-C3-MINI-1_V1.ipt
- D:\Projects\WearableWLED\WearableWLED_Mechanical\board\WearableWLED_Hardware\WearableWLED_Hardware\uid__1-191^DesignRootModel_PCB_ESP32-C3-MINI-1_V1(2)_PCB_ESP32-C3-MINI-1_V1.ipt
- D:\Projects\WearableWLED\WearableWLED_Mechanical\board\WearableWLED_Hardware\WearableWLED_Hardware\uid__1-192^DesignRootModel_PCB_ESP32-C3-MINI-1_V1(2)_PCB_ESP32-C3-MINI-1_V1.ipt
- D:\Projects\WearableWLED\WearableWLED_Mechanical\board\WearableWLED_Hardware\WearableWLED_Hardware\uid__1-193^DesignRootModel_PCB_ESP32-C3-MINI-1_V1(2)_PCB_ESP32-C3-MINI-1_V1.ipt
- D:\Projects\WearableWLED\WearableWLED_Mechanical\board\WearableWLED_Hardware\WearableWLED_Hardware\uid__1-194^DesignRootModel_PCB_ESP32-C3-MINI-1_V1(2)_PCB_ESP32-C3-MINI-1_V1.ipt
- D:\Projects\WearableWLED\WearableWLED_Mechanical\board\WearableWLED_Hardware\WearableWLED_Hardware\uid__1-195^DesignRootModel_PCB_ESP32-C3-MINI-1_V1(2)_PCB_ESP32-C3-MINI-1_V1.ipt
- D:\Projects\WearableWLED\WearableWLED_Mechanical\board\WearableWLED_Hardware\WearableWLED_Hardware\uid__1-196^DesignRootModel_PCB_ESP32-C3-MINI-1_V1(2)_PCB_ESP32-C3-MINI-1_V1.ipt
- D:\Projects\WearableWLED\WearableWLED_Mechanical\board\WearableWLED_Hardware\WearableWLED_Hardware\uid__1-197^DesignRootModel_PCB_ESP32-C3-MINI-1_V1(2)_PCB_ESP32-C3-MINI-1_V1.ipt
- D:\Projects\WearableWLED\WearableWLED_Mechanical\board\WearableWLED_Hardware\WearableWLED_Hardware\uid__1-198^DesignRootModel_PCB_ESP32-C3-MINI-1_V1(2)_PCB_ESP32-C3-MINI-1_V1.ipt
- D:\Projects\WearableWLED\WearableWLED_Mechanical\board\WearableWLED_Hardware\WearableWLED_Hardware\uid__1-199^DesignRootModel_PCB_ESP32-C3-MINI-1_V1(2)_PCB_ESP32-C3-MINI-1_V1.ipt
- D:\Projects\WearableWLED\WearableWLED_Mechanical\board\WearableWLED_Hardware\WearableWLED_Hardware\uid__1-200^DesignRootModel_PCB_ESP32-C3-MINI-1_V1(2)_PCB_ESP32-C3-MINI-1_V1.ipt
- D:\Projects\WearableWLED\WearableWLED_Mechanical\board\WearableWLED_Hardware\WearableWLED_Hardware\uid__1-201^DesignRootModel_PCB_ESP32-C3-MINI-1_V1(2)_PCB_ESP32-C3-MINI-1_V1.ipt
- D:\Projects\WearableWLED\WearableWLED_Mechanical\board\WearableWLED_Hardware\WearableWLED_Hardware\uid__1-202^DesignRootModel_PCB_ESP32-C3-MINI-1_V1(2)_PCB_ESP32-C3-MINI-1_V1.ipt